# Autodesk Inventor assembly: Core{XY}.old
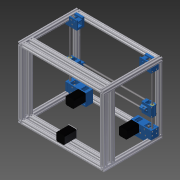
[picture p0: Inventor's stored thumbnail of the model, 180x180]
Saved by Autodesk Inventor 2015 (Build 190159000, 159)
## iProperties
Created: 2014-08-02
Part Number: Core{XY}.old
Document SubType Name: Assembly
Designer: Jack
Author: Jack
## Documents named in this file (11)
- C:\Users\t_clevj\ownCloud\CoreXY\InventorModel\Old\Core{XY}.old.iam
- C:\Users\t_clevj\ownCloud\CoreXY\InventorModel\Frame\Frame.iam
- C:\Users\t_clevj\ownCloud\CoreXY\InventorModel\Hardware\Shaft\Shaft8\Shaft8x310.old.ipt
- C:\Users\t_clevj\ownCloud\CoreXY\InventorModel\Old\YAxis\YAxisMotor\YAxisMotorLeft.old.iam
- C:\Users\t_clevj\ownCloud\CoreXY\InventorModel\Old\YAxis\YAxisIdler\YAxisIdlerLeft.old.iam
- C:\Users\t_clevj\ownCloud\CoreXY\InventorModel\Old\YAxis\YAxisMotor\YAxisMotorRight.old.iam
- C:\Users\t_clevj\ownCloud\CoreXY\InventorModel\Old\YAxis\YAxisIdler\YAxisIdlerRight.old.iam
- C:\Users\t_clevj\ownCloud\CoreXY\InventorModel\Hardware\Shaft\Shaft8\Shaft8x396.old.ipt
- C:\Users\t_clevj\ownCloud\CoreXY\InventorModel\Old\XAxis\XEndVert\XEndVertRight.old.iam
- C:\Users\t_clevj\ownCloud\CoreXY\InventorModel\Old\XAxis\XEndVert\XEndVertLeft.old.iam
- C:\Users\t_clevj\ownCloud\CoreXY\InventorModel\Old\ZAxis\ZMotor.old.iam
## Components (12 placed, 11 different names)
1. Frame:1 [sub-assembly] — Mate:1, Flush:1, Mate:2, Mate:41, Mate:42, Mate:43, Mate:44, Mate:45, Mate:46, Mate:50, Mate:51, Mate:52, Mate:53, Mate:54, Mate:55, Mate:71, Mate:72, Mate:73
2. ZMotor.old:1 [sub-assembly] — Mate:71, Mate:72, Mate:73
3. YAxisMotorLeft.old:1 [sub-assembly] — Mate:41, Mate:42, Mate:43, Mate:49, Mate:68
4. YAxisIdlerLeft.old:1 [sub-assembly] — Mate:44, Mate:45, Mate:46
5. Shaft8x310.old:1 — Mate:49, Mate:68, Mate:69
6. Shaft8x310.old:2 — Mate:56, Mate:58, Mate:65
7. YAxisIdlerRight.old:1 [sub-assembly] — Mate:51, Mate:52, Mate:55, Mate:58
8. YAxisMotorRight.old:1 [sub-assembly] — Mate:50, Mate:53, Mate:54, Mate:56
9. XEndVertLeft.old:1 [sub-assembly] — Mate:63, Mate:66, Mate:69
10. XEndVertRight.old:1 [sub-assembly] — Mate:61, Mate:62, Flush:2, Flush:3, Mate:65
11. XAxisRodBottom — Mate:62, Flush:2, Mate:66
12. XAxisRodTop — Mate:61, Flush:3, Mate:63
## Relationships (30: Mate 27, Flush 3)
- Mate:1: Frame:1
- Flush:1: Frame:1
- Mate:2: Frame:1
- Mate:41: Frame:1 ↔ YAxisMotorLeft.old:1
- Mate:42: Frame:1 ↔ YAxisMotorLeft.old:1
- Mate:43: Frame:1 ↔ YAxisMotorLeft.old:1
- Mate:44: Frame:1 ↔ YAxisIdlerLeft.old:1
- Mate:45: Frame:1 ↔ YAxisIdlerLeft.old:1
- Mate:46: Frame:1 ↔ YAxisIdlerLeft.old:1
- Mate:49: YAxisMotorLeft.old:1 ↔ Shaft8x310.old:1
- Mate:50: Frame:1 ↔ YAxisMotorRight.old:1
- Mate:51: Frame:1 ↔ YAxisIdlerRight.old:1
- Mate:52: Frame:1 ↔ YAxisIdlerRight.old:1
- Mate:53: Frame:1 ↔ YAxisMotorRight.old:1
- Mate:54: Frame:1 ↔ YAxisMotorRight.old:1
- Mate:55: Frame:1 ↔ YAxisIdlerRight.old:1
- Mate:56: Shaft8x310.old:2 ↔ YAxisMotorRight.old:1
- Mate:58: Shaft8x310.old:2 ↔ YAxisIdlerRight.old:1
- Mate:61: XEndVertRight.old:1 ↔ XAxisRodTop
- Mate:62: XEndVertRight.old:1 ↔ XAxisRodBottom
- Flush:2: XEndVertRight.old:1 ↔ XAxisRodBottom
- Flush:3: XEndVertRight.old:1 ↔ XAxisRodTop
- Mate:63: XEndVertLeft.old:1 ↔ XAxisRodTop
- Mate:65: Shaft8x310.old:2 ↔ XEndVertRight.old:1
- Mate:66: XEndVertLeft.old:1 ↔ XAxisRodBottom
- Mate:68: YAxisMotorLeft.old:1 ↔ Shaft8x310.old:1
- Mate:69: Shaft8x310.old:1 ↔ XEndVertLeft.old:1
- Mate:71 (178.85 mm): Frame:1 ↔ ZMotor.old:1
- Mate:72: Frame:1 ↔ ZMotor.old:1
- Mate:73: Frame:1 ↔ ZMotor.old:1
